# Autodesk Inventor assembly: gearLockAssembly
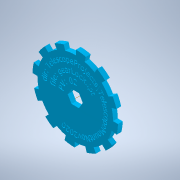
[picture p0: Inventor's stored thumbnail of the model, 180x180]
Saved by Autodesk Inventor 2021.2 (Build 252289000, 289)
## iProperties
Created: 2021-03-15
Part Number: gearLockAssembly
Document SubType Name: Assembly
Designer: robst
Author: robst
## Documents named in this file (3)
- C:\git\CAD-Development\robSteele\ShapeWays\TelescopeProjects\TelescopeMountNov2020\gearLockAssembly.iam
- C:\git\CAD-Development\robSteele\ShapeWays\TelescopeProjects\TelescopeMountNov2020\gearLockTopHalf.ipt
- C:\Users\robst\Documents\Inventor\Content Center Files\R2021\en-US\ANSI B18.3(03)\ANSI B18.3 - 10-32 UNF - UNF - 1(1).ipt
## Components (2 placed, 2 different names)
1. gearLockTopHalf:1 — Flush:1
2. Hexagon Socket Button Head Cap Screw - Inch No. 10-32 - 1:1 — Flush:1
## Relationships (1: Flush 1)
- Flush:1: gearLockTopHalf:1 ↔ Hexagon Socket Button Head Cap Screw - Inch No. 10-32 - 1:1
